# Autodesk Inventor assembly: version entrega 2
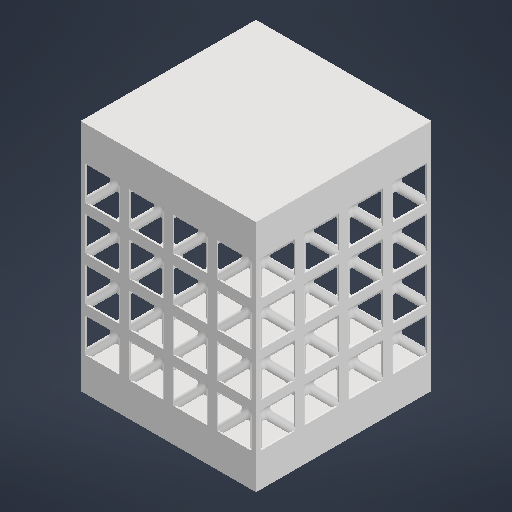
[picture p0: Inventor's stored thumbnail of the model, 512x512]
Saved by Autodesk Inventor 2026.1 (Build 301233020, 233B)
## iProperties
Created: 2025-11-13
Part Number: version entrega 2
Document SubType Name: Assembly
Designer: benja
Author: benja
## Documents named in this file (3)
- C:\Users\benja\OneDrive\Escritorio\version entrega 2.iam
- C:\Users\benja\OneDrive\Escritorio\Placa entrega 2.ipt
- C:\Users\benja\OneDrive\Escritorio\Patron BBC entrega 2.ipt
## Components (66 placed, 2 different names)
1. Placa entrega 2:1 — Coincidencia:1, Coincidencia:2, Coincidencia:3, Coincidencia:4, Nivelación:1, Nivelación:2, Nivelación:3, Nivelación:4, Nivelación:5, Nivelación:6, Coincidencia:8, Coincidencia:9, Coincidencia:10, Coincidencia:11, Coincidencia:12, Coincidencia:13, Coincidencia:14, Nivelación:7, Nivelación:8, Nivelación:9, Nivelación:10, Coincidencia:25, Coincidencia:26, Coincidencia:27, Coincidencia:28, Coincidencia:29, Nivelación:11, Nivelación:12, Nivelación:13
2. Patron BBC entrega 2:1 — Coincidencia:11, Coincidencia:19, Coincidencia:21, Coincidencia:34
3. Patron BBC entrega 2:2 — Coincidencia:3, Coincidencia:6, Nivelación:4, Coincidencia:7, Coincidencia:19, Nivelación:40
4. Patron BBC entrega 2:3 — Coincidencia:10, Coincidencia:18, Coincidencia:20, Coincidencia:21, Coincidencia:24
5. Patron BBC entrega 2:4 — Coincidencia:14, Nivelación:7, Coincidencia:15, Coincidencia:16, Coincidencia:20, Nivelación:36
6. Patron BBC entrega 2:5 — Coincidencia:8, Coincidencia:23, Coincidencia:24, Coincidencia:31
7. Patron BBC entrega 2:6 — Coincidencia:13, Nivelación:9, Coincidencia:17, Coincidencia:30, Nivelación:14, Coincidencia:75, Nivelación:15, Nivelación:34
8. Patron BBC entrega 2:7 — Coincidencia:9, Nivelación:8, Coincidencia:15, Coincidencia:17, Coincidencia:23, Nivelación:35
9. Patron BBC entrega 2:8 — Coincidencia:2, Nivelación:1, Nivelación:2, Coincidencia:5, Coincidencia:16, Nivelación:37, Nivelación:39
10. Patron BBC entrega 2:9 — Coincidencia:4, Nivelación:5, Coincidencia:7, Nivelación:6, Coincidencia:22, Nivelación:41
11. Patron BBC entrega 2:10 — Coincidencia:1, Nivelación:3, Coincidencia:5, Coincidencia:6, Coincidencia:18, Nivelación:38
12. Patron BBC entrega 2:11 — Coincidencia:26, Coincidencia:33, Nivelación:13, Coincidencia:37, Nivelación:31, Nivelación:42
13. Patron BBC entrega 2:12 — Coincidencia:12, Coincidencia:22, Nivelación:10, Coincidencia:32, Nivelación:44
14. Patron BBC entrega 2:13 — Coincidencia:28, Coincidencia:32, Nivelación:12, Coincidencia:33, Coincidencia:35, Nivelación:43
15. Patron BBC entrega 2:14 — Coincidencia:25, Coincidencia:30, Coincidencia:31, Nivelación:11, Nivelación:33
16. Patron BBC entrega 2:15 — Coincidencia:27, Coincidencia:36, Coincidencia:37, Nivelación:32
17. Patron BBC entrega 2:16 — Coincidencia:29, Coincidencia:34, Coincidencia:35, Coincidencia:36
18. Patron BBC entrega 2:17 — Nivelación:45, Nivelación:46, Nivelación:48, Nivelación:59
19. Patron BBC entrega 2:18 — Nivelación:40, Nivelación:59, Nivelación:60
20. Patron BBC entrega 2:19 — Nivelación:48, Nivelación:57
21. Patron BBC entrega 2:20 — Nivelación:36, Nivelación:56
22. Patron BBC entrega 2:21 — Nivelación:47
23. Patron BBC entrega 2:22 — Nivelación:14, Coincidencia:75, Nivelación:15, Nivelación:34, Nivelación:51, Nivelación:55
24. Patron BBC entrega 2:23 — Nivelación:35, Nivelación:55, Nivelación:56
25. Patron BBC entrega 2:24 — Nivelación:37, Nivelación:39, Nivelación:57, Nivelación:58
26. Patron BBC entrega 2:25 — Nivelación:41, Nivelación:61, Nivelación:62, Nivelación:63
27. Patron BBC entrega 2:26 — Nivelación:38, Nivelación:58, Nivelación:60
28. Patron BBC entrega 2:27 — Nivelación:31, Nivelación:42, Nivelación:49, Nivelación:50, Nivelación:53, Coincidencia:135
29. Patron BBC entrega 2:28 — Nivelación:44, Nivelación:45, Nivelación:61
30. Patron BBC entrega 2:29 — Nivelación:43, Nivelación:49, Nivelación:54
31. Patron BBC entrega 2:30 — Nivelación:33, Nivelación:51, Nivelación:52
32. Patron BBC entrega 2:31 — Nivelación:32, Nivelación:50, Nivelación:52, Nivelación:53
33. Patron BBC entrega 2:32 — Nivelación:46, Nivelación:47, Nivelación:54
34. Placa entrega 2:3
35. Patron BBC entrega 2:33
36. Patron BBC entrega 2:34
37. Patron BBC entrega 2:35
38. Patron BBC entrega 2:36
39. Patron BBC entrega 2:37
40. Patron BBC entrega 2:38
41. Patron BBC entrega 2:39
42. Patron BBC entrega 2:40
43. Patron BBC entrega 2:41
44. Patron BBC entrega 2:42
45. Patron BBC entrega 2:43
46. Patron BBC entrega 2:44
47. Patron BBC entrega 2:45
48. Patron BBC entrega 2:46
49. Patron BBC entrega 2:47
50. Patron BBC entrega 2:48
51. Patron BBC entrega 2:49
52. Patron BBC entrega 2:50
53. Patron BBC entrega 2:51
54. Patron BBC entrega 2:52 — Coincidencia:135
55. Patron BBC entrega 2:53
56. Patron BBC entrega 2:54
57. Patron BBC entrega 2:55
58. Patron BBC entrega 2:56
59. Patron BBC entrega 2:57
60. Patron BBC entrega 2:58
61. Patron BBC entrega 2:59 — Nivelación:62, Nivelación:63
62. Patron BBC entrega 2:60
63. Patron BBC entrega 2:61
64. Patron BBC entrega 2:62
65. Patron BBC entrega 2:63
66. Patron BBC entrega 2:64
## Relationships (182: Mate 119, Flush 63)
- Coincidencia:1 [Mate]: Placa entrega 2:1 ↔ Patron BBC entrega 2:10
- Coincidencia:2 [Mate]: Placa entrega 2:1 ↔ Patron BBC entrega 2:8
- Coincidencia:3 [Mate]: Placa entrega 2:1 ↔ Patron BBC entrega 2:2
- Coincidencia:4 [Mate]: Placa entrega 2:1 ↔ Patron BBC entrega 2:9
- Nivelación:1 [Flush]: Placa entrega 2:1 ↔ Patron BBC entrega 2:8
- Nivelación:2 [Flush]: Placa entrega 2:1 ↔ Patron BBC entrega 2:8
- Nivelación:3 [Flush]: Placa entrega 2:1 ↔ Patron BBC entrega 2:10
- Coincidencia:5 [Mate]: Patron BBC entrega 2:8 ↔ Patron BBC entrega 2:10
- Coincidencia:6 [Mate]: Patron BBC entrega 2:2 ↔ Patron BBC entrega 2:10
- Nivelación:4 [Flush]: Placa entrega 2:1 ↔ Patron BBC entrega 2:2
- Nivelación:5 [Flush]: Placa entrega 2:1 ↔ Patron BBC entrega 2:9
- Coincidencia:7 [Mate]: Patron BBC entrega 2:2 ↔ Patron BBC entrega 2:9
- Nivelación:6 [Flush]: Placa entrega 2:1 ↔ Patron BBC entrega 2:9
- Coincidencia:8 [Mate]: Placa entrega 2:1 ↔ Patron BBC entrega 2:5
- Coincidencia:9 [Mate]: Placa entrega 2:1 ↔ Patron BBC entrega 2:7
- Coincidencia:10 [Mate]: Placa entrega 2:1 ↔ Patron BBC entrega 2:3
- Coincidencia:11 [Mate]: Placa entrega 2:1 ↔ Patron BBC entrega 2:1
- Coincidencia:12 [Mate]: Placa entrega 2:1 ↔ Patron BBC entrega 2:12
- Coincidencia:13 [Mate]: Placa entrega 2:1 ↔ Patron BBC entrega 2:6
- Coincidencia:14 [Mate]: Placa entrega 2:1 ↔ Patron BBC entrega 2:4
- Nivelación:7 [Flush]: Placa entrega 2:1 ↔ Patron BBC entrega 2:4
- Nivelación:8 [Flush]: Placa entrega 2:1 ↔ Patron BBC entrega 2:7
- Coincidencia:15 [Mate]: Patron BBC entrega 2:4 ↔ Patron BBC entrega 2:7
- Coincidencia:16 [Mate]: Patron BBC entrega 2:4 ↔ Patron BBC entrega 2:8
- Nivelación:9 [Flush]: Placa entrega 2:1 ↔ Patron BBC entrega 2:6
- Coincidencia:17 [Mate]: Patron BBC entrega 2:6 ↔ Patron BBC entrega 2:7
- Coincidencia:18 [Mate]: Patron BBC entrega 2:3 ↔ Patron BBC entrega 2:10
- Coincidencia:19 [Mate]: Patron BBC entrega 2:1 ↔ Patron BBC entrega 2:2
- Coincidencia:20 [Mate]: Patron BBC entrega 2:3 ↔ Patron BBC entrega 2:4
- Coincidencia:21 [Mate]: Patron BBC entrega 2:1 ↔ Patron BBC entrega 2:3
- Coincidencia:22 [Mate]: Patron BBC entrega 2:9 ↔ Patron BBC entrega 2:12
- Nivelación:10 [Flush]: Placa entrega 2:1 ↔ Patron BBC entrega 2:12
- Coincidencia:23 [Mate]: Patron BBC entrega 2:5 ↔ Patron BBC entrega 2:7
- Coincidencia:24 [Mate]: Patron BBC entrega 2:3 ↔ Patron BBC entrega 2:5
- Coincidencia:25 [Mate]: Placa entrega 2:1 ↔ Patron BBC entrega 2:14
- Coincidencia:26 [Mate]: Placa entrega 2:1 ↔ Patron BBC entrega 2:11
- Coincidencia:27 [Mate]: Placa entrega 2:1 ↔ Patron BBC entrega 2:15
- Coincidencia:28 [Mate]: Placa entrega 2:1 ↔ Patron BBC entrega 2:13
- Coincidencia:29 [Mate]: Placa entrega 2:1 ↔ Patron BBC entrega 2:16
- Coincidencia:30 [Mate]: Patron BBC entrega 2:6 ↔ Patron BBC entrega 2:14
- Coincidencia:31 [Mate]: Patron BBC entrega 2:5 ↔ Patron BBC entrega 2:14
- Nivelación:11 [Flush]: Placa entrega 2:1 ↔ Patron BBC entrega 2:14
- Coincidencia:32 [Mate]: Patron BBC entrega 2:12 ↔ Patron BBC entrega 2:13
- Nivelación:12 [Flush]: Placa entrega 2:1 ↔ Patron BBC entrega 2:13
- Coincidencia:33 [Mate]: Patron BBC entrega 2:11 ↔ Patron BBC entrega 2:13
- Nivelación:13 [Flush]: Placa entrega 2:1 ↔ Patron BBC entrega 2:11
- Coincidencia:34 [Mate]: Patron BBC entrega 2:1 ↔ Patron BBC entrega 2:16
- Coincidencia:35 [Mate]: Patron BBC entrega 2:13 ↔ Patron BBC entrega 2:16
- Coincidencia:36 [Mate]: Patron BBC entrega 2:15 ↔ Patron BBC entrega 2:16
- Coincidencia:37 [Mate]: Patron BBC entrega 2:11 ↔ Patron BBC entrega 2:15
- [Mate]: Patron BBC entrega 2:24 ↔ Patron BBC entrega 2:26
- [Mate]: Patron BBC entrega 2:18 ↔ Patron BBC entrega 2:26
- [Mate]: Patron BBC entrega 2:18 ↔ Patron BBC entrega 2:25
- [Mate]: Patron BBC entrega 2:20 ↔ Patron BBC entrega 2:23
- [Mate]: Patron BBC entrega 2:20 ↔ Patron BBC entrega 2:24
- [Mate]: Patron BBC entrega 2:22 ↔ Patron BBC entrega 2:23
- [Mate]: Patron BBC entrega 2:19 ↔ Patron BBC entrega 2:26
- [Mate]: Patron BBC entrega 2:17 ↔ Patron BBC entrega 2:18
- [Mate]: Patron BBC entrega 2:19 ↔ Patron BBC entrega 2:20
- [Mate]: Patron BBC entrega 2:17 ↔ Patron BBC entrega 2:19
- [Mate]: Patron BBC entrega 2:25 ↔ Patron BBC entrega 2:28
- [Mate]: Patron BBC entrega 2:21 ↔ Patron BBC entrega 2:23
- [Mate]: Patron BBC entrega 2:19 ↔ Patron BBC entrega 2:21
- [Mate]: Patron BBC entrega 2:22 ↔ Patron BBC entrega 2:30
- [Mate]: Patron BBC entrega 2:21 ↔ Patron BBC entrega 2:30
- [Mate]: Patron BBC entrega 2:28 ↔ Patron BBC entrega 2:29
- [Mate]: Patron BBC entrega 2:27 ↔ Patron BBC entrega 2:29
- [Mate]: Patron BBC entrega 2:17 ↔ Patron BBC entrega 2:32
- [Mate]: Patron BBC entrega 2:29 ↔ Patron BBC entrega 2:32
- [Mate]: Patron BBC entrega 2:31 ↔ Patron BBC entrega 2:32
- [Mate]: Patron BBC entrega 2:27 ↔ Patron BBC entrega 2:31
- Nivelación:14 [Flush]: Patron BBC entrega 2:6 ↔ Patron BBC entrega 2:22
- Coincidencia:75 [Mate]: Patron BBC entrega 2:6 ↔ Patron BBC entrega 2:22
- Nivelación:15 [Flush]: Patron BBC entrega 2:6 ↔ Patron BBC entrega 2:22
- [Mate]: Placa entrega 2:3 ↔ Patron BBC entrega 2:42
- [Mate]: Placa entrega 2:3 ↔ Patron BBC entrega 2:40
- [Mate]: Placa entrega 2:3 ↔ Patron BBC entrega 2:34
- [Mate]: Placa entrega 2:3 ↔ Patron BBC entrega 2:41
- [Flush]: Placa entrega 2:3 ↔ Patron BBC entrega 2:40
- [Flush]: Placa entrega 2:3 ↔ Patron BBC entrega 2:40
- [Flush]: Placa entrega 2:3 ↔ Patron BBC entrega 2:42
- [Mate]: Patron BBC entrega 2:40 ↔ Patron BBC entrega 2:42
- [Mate]: Patron BBC entrega 2:34 ↔ Patron BBC entrega 2:42
- [Flush]: Placa entrega 2:3 ↔ Patron BBC entrega 2:34
- [Flush]: Placa entrega 2:3 ↔ Patron BBC entrega 2:41
- [Mate]: Patron BBC entrega 2:34 ↔ Patron BBC entrega 2:41
- [Flush]: Placa entrega 2:3 ↔ Patron BBC entrega 2:41
- [Mate]: Placa entrega 2:3 ↔ Patron BBC entrega 2:37
- [Mate]: Placa entrega 2:3 ↔ Patron BBC entrega 2:39
- [Mate]: Placa entrega 2:3 ↔ Patron BBC entrega 2:35
- [Mate]: Placa entrega 2:3 ↔ Patron BBC entrega 2:33
- [Mate]: Placa entrega 2:3 ↔ Patron BBC entrega 2:44
- [Mate]: Placa entrega 2:3 ↔ Patron BBC entrega 2:38
- [Mate]: Placa entrega 2:3 ↔ Patron BBC entrega 2:36
- [Flush]: Placa entrega 2:3 ↔ Patron BBC entrega 2:36
- [Flush]: Placa entrega 2:3 ↔ Patron BBC entrega 2:39
- [Mate]: Patron BBC entrega 2:36 ↔ Patron BBC entrega 2:39
- [Mate]: Patron BBC entrega 2:36 ↔ Patron BBC entrega 2:40
- [Flush]: Placa entrega 2:3 ↔ Patron BBC entrega 2:38
- [Mate]: Patron BBC entrega 2:38 ↔ Patron BBC entrega 2:39
- [Mate]: Patron BBC entrega 2:35 ↔ Patron BBC entrega 2:42
- [Mate]: Patron BBC entrega 2:33 ↔ Patron BBC entrega 2:34
- [Mate]: Patron BBC entrega 2:35 ↔ Patron BBC entrega 2:36
- [Mate]: Patron BBC entrega 2:33 ↔ Patron BBC entrega 2:35
- [Mate]: Patron BBC entrega 2:41 ↔ Patron BBC entrega 2:44
- [Flush]: Placa entrega 2:3 ↔ Patron BBC entrega 2:44
- [Mate]: Patron BBC entrega 2:37 ↔ Patron BBC entrega 2:39
- [Mate]: Patron BBC entrega 2:35 ↔ Patron BBC entrega 2:37
- [Mate]: Placa entrega 2:3 ↔ Patron BBC entrega 2:46
- [Mate]: Placa entrega 2:3 ↔ Patron BBC entrega 2:43
- [Mate]: Placa entrega 2:3 ↔ Patron BBC entrega 2:47
- [Mate]: Placa entrega 2:3 ↔ Patron BBC entrega 2:45
- [Mate]: Placa entrega 2:3 ↔ Patron BBC entrega 2:48
- [Mate]: Patron BBC entrega 2:38 ↔ Patron BBC entrega 2:46
- [Mate]: Patron BBC entrega 2:37 ↔ Patron BBC entrega 2:46
- [Flush]: Placa entrega 2:3 ↔ Patron BBC entrega 2:46
- [Mate]: Patron BBC entrega 2:44 ↔ Patron BBC entrega 2:45
- [Flush]: Placa entrega 2:3 ↔ Patron BBC entrega 2:45
- [Mate]: Patron BBC entrega 2:43 ↔ Patron BBC entrega 2:45
- [Flush]: Placa entrega 2:3 ↔ Patron BBC entrega 2:43
- [Mate]: Patron BBC entrega 2:33 ↔ Patron BBC entrega 2:48
- [Mate]: Patron BBC entrega 2:45 ↔ Patron BBC entrega 2:48
- [Mate]: Patron BBC entrega 2:47 ↔ Patron BBC entrega 2:48
- [Mate]: Patron BBC entrega 2:43 ↔ Patron BBC entrega 2:47
- [Mate]: Patron BBC entrega 2:56 ↔ Patron BBC entrega 2:58
- [Mate]: Patron BBC entrega 2:50 ↔ Patron BBC entrega 2:58
- [Mate]: Patron BBC entrega 2:50 ↔ Patron BBC entrega 2:57
- [Mate]: Patron BBC entrega 2:52 ↔ Patron BBC entrega 2:55
- [Mate]: Patron BBC entrega 2:52 ↔ Patron BBC entrega 2:56
- [Mate]: Patron BBC entrega 2:54 ↔ Patron BBC entrega 2:55
- [Mate]: Patron BBC entrega 2:51 ↔ Patron BBC entrega 2:58
- [Mate]: Patron BBC entrega 2:49 ↔ Patron BBC entrega 2:50
- [Mate]: Patron BBC entrega 2:51 ↔ Patron BBC entrega 2:52
- [Mate]: Patron BBC entrega 2:49 ↔ Patron BBC entrega 2:51
- [Mate]: Patron BBC entrega 2:57 ↔ Patron BBC entrega 2:60
- [Mate]: Patron BBC entrega 2:53 ↔ Patron BBC entrega 2:55
- [Mate]: Patron BBC entrega 2:51 ↔ Patron BBC entrega 2:53
- [Mate]: Patron BBC entrega 2:54 ↔ Patron BBC entrega 2:62
- [Mate]: Patron BBC entrega 2:53 ↔ Patron BBC entrega 2:62
- [Mate]: Patron BBC entrega 2:60 ↔ Patron BBC entrega 2:61
- [Mate]: Patron BBC entrega 2:59 ↔ Patron BBC entrega 2:61
- [Mate]: Patron BBC entrega 2:49 ↔ Patron BBC entrega 2:64
- [Mate]: Patron BBC entrega 2:61 ↔ Patron BBC entrega 2:64
- [Mate]: Patron BBC entrega 2:63 ↔ Patron BBC entrega 2:64
- [Mate]: Patron BBC entrega 2:59 ↔ Patron BBC entrega 2:63
- [Flush]: Patron BBC entrega 2:38 ↔ Patron BBC entrega 2:54
- [Mate]: Patron BBC entrega 2:38 ↔ Patron BBC entrega 2:54
- [Flush]: Patron BBC entrega 2:38 ↔ Patron BBC entrega 2:54
- Nivelación:31 [Flush]: Patron BBC entrega 2:11 ↔ Patron BBC entrega 2:27
- Nivelación:32 [Flush]: Patron BBC entrega 2:15 ↔ Patron BBC entrega 2:31
- Nivelación:33 [Flush]: Patron BBC entrega 2:14 ↔ Patron BBC entrega 2:30
- Nivelación:34 [Flush]: Patron BBC entrega 2:6 ↔ Patron BBC entrega 2:22
- Nivelación:35 [Flush]: Patron BBC entrega 2:7 ↔ Patron BBC entrega 2:23
- Nivelación:36 [Flush]: Patron BBC entrega 2:4 ↔ Patron BBC entrega 2:20
- Nivelación:37 [Flush]: Patron BBC entrega 2:8 ↔ Patron BBC entrega 2:24
- Nivelación:38 [Flush]: Patron BBC entrega 2:10 ↔ Patron BBC entrega 2:26
- Nivelación:39 [Flush]: Patron BBC entrega 2:8 ↔ Patron BBC entrega 2:24
- Nivelación:40 [Flush]: Patron BBC entrega 2:2 ↔ Patron BBC entrega 2:18
- Nivelación:41 [Flush]: Patron BBC entrega 2:9 ↔ Patron BBC entrega 2:25
- Nivelación:42 [Flush]: Patron BBC entrega 2:11 ↔ Patron BBC entrega 2:27
- Nivelación:43 [Flush]: Patron BBC entrega 2:13 ↔ Patron BBC entrega 2:29
- Nivelación:44 [Flush]: Patron BBC entrega 2:12 ↔ Patron BBC entrega 2:28
- Nivelación:45 [Flush]: Patron BBC entrega 2:17 ↔ Patron BBC entrega 2:28
- Nivelación:46 [Flush]: Patron BBC entrega 2:17 ↔ Patron BBC entrega 2:32
- Nivelación:47 [Flush]: Patron BBC entrega 2:21 ↔ Patron BBC entrega 2:32
- Nivelación:48 [Flush]: Patron BBC entrega 2:17 ↔ Patron BBC entrega 2:19
- Nivelación:49 [Flush]: Patron BBC entrega 2:27 ↔ Patron BBC entrega 2:29
- Nivelación:50 [Flush]: Patron BBC entrega 2:27 ↔ Patron BBC entrega 2:31
- Nivelación:51 [Flush]: Patron BBC entrega 2:22 ↔ Patron BBC entrega 2:30
- Nivelación:52 [Flush]: Patron BBC entrega 2:30 ↔ Patron BBC entrega 2:31
- Nivelación:53 [Flush]: Patron BBC entrega 2:27 ↔ Patron BBC entrega 2:31
- Nivelación:54 [Flush]: Patron BBC entrega 2:29 ↔ Patron BBC entrega 2:32
- Nivelación:55 [Flush]: Patron BBC entrega 2:22 ↔ Patron BBC entrega 2:23
- Nivelación:56 [Flush]: Patron BBC entrega 2:20 ↔ Patron BBC entrega 2:23
- Nivelación:57 [Flush]: Patron BBC entrega 2:19 ↔ Patron BBC entrega 2:24
- Nivelación:58 [Flush]: Patron BBC entrega 2:24 ↔ Patron BBC entrega 2:26
- Nivelación:59 [Flush]: Patron BBC entrega 2:17 ↔ Patron BBC entrega 2:18
- Nivelación:60 [Flush]: Patron BBC entrega 2:18 ↔ Patron BBC entrega 2:26
- Nivelación:61 [Flush]: Patron BBC entrega 2:25 ↔ Patron BBC entrega 2:28
- Coincidencia:135 [Mate]: Patron BBC entrega 2:27 ↔ Patron BBC entrega 2:52
- Nivelación:62 [Flush]: Patron BBC entrega 2:25 ↔ Patron BBC entrega 2:59
- Nivelación:63 [Flush]: Patron BBC entrega 2:25 ↔ Patron BBC entrega 2:59
## Named parameters: d59_d22 = 0 mm, d60_d23 = 0 mm, d62_d25 = 0 mm, d63_d26 = 0 mm, d64_d27 = 0 mm, d65_d28 = 0 mm, d66_d29 = 0 mm, d67_d30 = 0 mm, d69_d32 = 0 mm, d70_d33 = 0 mm, d76_d39 = 0 mm, d77_d40 = 0 mm, d79_d42 = 0 mm, d81_d44 = 0 mm, d83_d46 = 0 mm, d84_d47 = 0 mm, d85_d48 = 0 mm, d86_d49 = 0 mm, d92_d7 = 0 mm, d93_d8 = 0 mm, d96_d11 = 0 mm, d103_d0 = 0 mm, d104_d1 = 0 mm, d105_d102 = 0 mm, d106_d69_d32 = 0 mm, d107_d70_d33 = 0 mm, d108_d76_d39 = 0 mm, d109_d77_d40 = 0 mm, d110_d79_d42 = 0 mm, d111_d81_d44 = 0 mm, d112_d83_d46 = 0 mm, d113_d84_d47 = 0 mm, d114_d85_d48 = 0 mm, d115_d86_d49 = 0 mm, d116_d92_d7 = 0 mm, d117_d93_d8 = 0 mm, d118_d96_d11 = 0 mm, d119_d100 = 0 mm, d120_d101 = 0 mm, d121_d15 = 0 mm, d122_d16 = 0 mm, d123_d17 = 0 mm, d124_d18 = 0 mm, d125_d19 = 0 mm, d126_d20 = 0 mm, d127_d21 = 0 mm, d128_d22 = 0 mm, d129_d23 = 0 mm, d130_d24 = 0 mm, d131_d25 = 0 mm, d132_d26 = 0 mm, d133_d27 = 0 mm, d134_d28 = 0 mm, d135_d29 = 0 mm, d136_d30 = 0 mm, d137_d31 = 0 mm, d138_d32 = 0 mm, d139_d33 = 0 mm, d140_d34 = 0 mm, d141_d35 = 0 mm, d142_d36 = 0 mm, d143_d37 = 0 mm, d144_d38 = 0 mm, d145_d39 = 0 mm, d146_d40 = 0 mm, d147_d41 = 0 mm, d148_d42 = 0 mm, d149_d43 = 0 mm, d150_d44 = 0 mm, d151_d45 = 0 mm, d152_d46 = 0 mm, d153_d47 = 0 mm, d154_d48 = 0 mm, d155_d49 = 0 mm, d156_d59_d22 = 0 mm, d157_d60_d23 = 0 mm, d158_d62_d25 = 0 mm, d159_d63_d26 = 0 mm, d160_d64_d27 = 0 mm, d161_d65_d28 = 0 mm, d162_d66_d29 = 0 mm, d163_d67_d30 = 0 mm, d164_d2 = 0 mm, d165_d3 = 0 mm, d166_d4 = 0 mm, d167_d5 = 0 mm, d168_d6 = 0 mm, d169_d7 = 0 mm, d170_d8 = 0 mm, d171_d9 = 0 mm, d172_d10 = 0 mm, d173_d11 = 0 mm, d174_d12 = 0 mm, d175_d13 = 0 mm, d176_d14 = 0 mm
